# Autodesk Inventor assembly: EL2-C-200
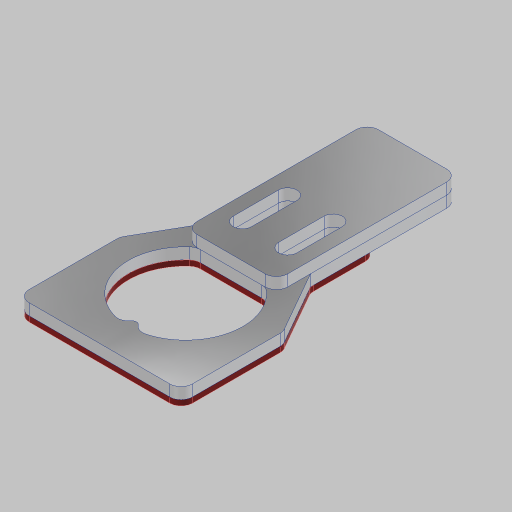
[picture p0: Inventor's stored thumbnail of the model, 512x512]
Saved by Autodesk Inventor 2023.5 (Build 275446000, 446)
## iProperties
Created: 2025-02-15
Part Number: EL2-C-200
Document SubType Name: Assembly
Designer: slick
Author: slick
## Documents named in this file (4)
- C:\Users\slick\OneDrive\Desktop\2025-ReefScape---CAD\Elevator\EL2\EL2-C-200.iam
- C:\Users\slick\OneDrive\Desktop\2025-ReefScape---CAD\Elevator\EL2\EL2-032.ipt
- C:\Users\slick\OneDrive\Desktop\2025-ReefScape---CAD\Elevator\EL2\EL2-C-006.ipt
- C:\Users\slick\OneDrive\Desktop\2025-ReefScape---CAD\Elevator\EL2\EL2-034.ipt
## Components (3 placed, 3 different names)
1. EL2-032:1 — Mate:1, Mate:2, Mate:3
2. EL2-C-006:1 — Mate:1, Mate:2, Mate:3, Mate:4, Mate:5, Mate:6
3. EL2-034:1 — Mate:4, Mate:5, Mate:6
## Relationships (6: Mate 6)
- Mate:1: EL2-032:1 ↔ EL2-C-006:1
- Mate:2: EL2-032:1 ↔ EL2-C-006:1
- Mate:3: EL2-032:1 ↔ EL2-C-006:1
- Mate:4: EL2-C-006:1 ↔ EL2-034:1
- Mate:5: EL2-C-006:1 ↔ EL2-034:1
- Mate:6: EL2-C-006:1 ↔ EL2-034:1
